# Autodesk Inventor assembly: PowerConnector
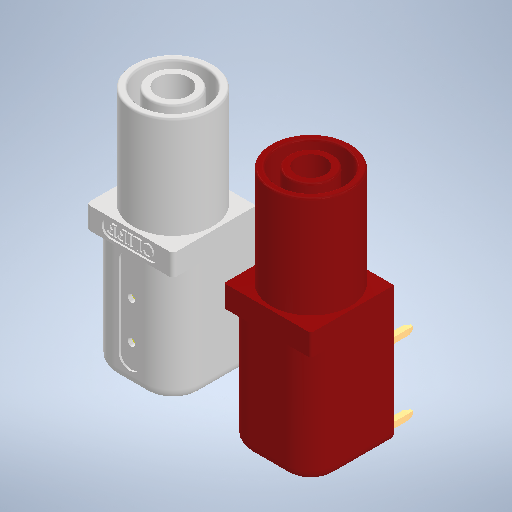
[picture p0: Inventor's stored thumbnail of the model, 512x512]
Saved by Autodesk Inventor 2025 (Build 290162000, 162)
## iProperties
Created: 2026-01-20
Part Number: PowerConnector
Document SubType Name: Assembly
Designer: tapen
Author: tapen
## Documents named in this file (3)
- C:\Users\tapen\OneDrive\Desktop\Chris Bidinosti\KVL+KCL\libs\3DModel\ipt\PowerConnector.iam
- C:\Users\tapen\OneDrive\Desktop\Chris Bidinosti\KVL+KCL\libs\FCR7350R\FCR7350\FCR7350.ipt
- C:\Users\tapen\OneDrive\Desktop\Chris Bidinosti\KVL+KCL\libs\FCR7350R\FCR7350R\FCR7350R.ipt
## Components (2 placed, 2 different names)
1. FCR7350:1 — Flush:1, Flush:2, Mate:1, Mate:2
2. FCR7350R:2 — Flush:1, Flush:2, Mate:1
## Relationships (4: Flush 2, Mate 2)
- Flush:1: FCR7350:1 ↔ FCR7350R:2
- Flush:2: FCR7350:1 ↔ FCR7350R:2
- Mate:1 (19.05 mm): FCR7350:1 ↔ FCR7350R:2
- Mate:2 (9.525 mm): FCR7350:1
